# Autodesk Inventor assembly: logitech_C90
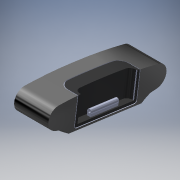
[picture p0: Inventor's stored thumbnail of the model, 180x180]
Saved by Autodesk Inventor 2019.3 (Build 233278000, 278)
## iProperties
Created: 2021-01-13
Part Number: logitech_C90
Material: Generisch
Document SubType Name: Assembly
Designer: Nicolas Frick
Author: Nicolas Frick
## Documents named in this file (2)
- C:\Users\Nicolas Frick\Sync\OneDrive\airhockeybot\mechanical_design\inventor\logitech_C90.iam
- C:\Users\Nicolas Frick\Sync\OneDrive\airhockeybot\mechanical_design\inventor\logitech\Logitech_C920.ipt
## Components (1 placed, 1 different names)
1. Logitech_C920:1 — Fluchtend:1, Passend:1
## Relationships (2: Flush 1, Mate 1)
- Fluchtend:1 [Flush] (-13.5 mm): Logitech_C920:1
- Passend:1 [Mate]: Logitech_C920:1
